# Autodesk Inventor assembly: Lift Assembly Right
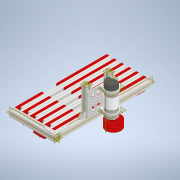
[picture p0: Inventor's stored thumbnail of the model, 180x180]
Saved by Autodesk Inventor 2020 (Build 240168000, 168)
## iProperties
Created: 2019-12-26
Part Number: Lift Assembly Right
Document SubType Name: Assembly
Designer: ball
Author: ball
## Documents named in this file (14)
- D:\FTC8863\2019 Robot\Delivery\Lift Right\Lift Assembly Right.iam
- D:\FTC8863\2019 Robot\Delivery\Lift Right\SAR330  x 5 + couplers right.iam
- D:\FTC8863\Actobotics\585 parts\585075.ipt
- D:\FTC8863\Actobotics\565 parts\xrail_3.5in.ipt
- D:\FTC8863\Actobotics\555 parts\555116 assembly.ipt
- D:\FTC8863\Actobotics\585 parts\585721.ipt
- D:\FTC8863\2019 Robot\Delivery\spool double 2 in diameter.iam
- D:\FTC8863\Andymark\am-2964a Neverest Classic 40.ipt
- D:\FTC8863\2019 Robot\Delivery\Lift Right\Limit switch top + mount right.iam
- D:\FTC8863\StepLibraries\Screws\M3 x 25 HEX HEAD CAP SCREW.ipt
- D:\FTC8863\2019 Robot\Delivery\Lift Right\Limit switch bottom + mount right.iam
- D:\FTC8863\Actobotics\585 parts\585071.ipt
- D:\FTC8863\2019 Robot\Delivery\x-rail 6.026 in.ipt
- D:\FTC8863\Actobotics\585 parts\585076.ipt
## Components (18 placed, 13 different names)
1. SAR330  x 5 + couplers right:1 [sub-assembly] — Mate:8, Flush:3, Mate:18, Mate:25, Mate:48, Mate:49, Flush:10, Mate:51, Mate:53, Flush:11, Mate:65, Flush:14, Mate:66, Mate:67, Mate:73, Mate:75, Flush:18
2. x-rail 6.026 in:1 — Mate:8, Flush:3, Mate:54, Mate:55, Mate:68, Mate:69, Mate:70
3. 585075:2
4. xrail_3.5in:2 — Flush:15, Flush:16, Mate:66, Mate:76, Mate:77, Flush:18
5. xrail_3.5in:3 — Mate:18, Mate:25, Mate:56, Flush:12, Mate:57, Flush:16, Mate:74, Flush:17
6. 585721:1 — Mate:57, Mate:58, Flush:13, Mate:59, Mate:61, Mate:62, Mate:65, Flush:15
7. 585721:2 — Mate:56, Flush:12, Mate:58, Flush:13, Mate:60, Mate:63, Mate:64
8. 555116 assembly:3 — Mate:46, Mate:59, Mate:61, Mate:62
9. 555116 assembly:4 — Mate:60, Mate:63, Mate:64
10. spool double 2 in diameter:1 [sub-assembly] — Flush:14
11. am-2964a Neverest Classic 40:1 — Mate:46
12. Limit switch top + mount right:1 [sub-assembly] — Mate:48, Mate:49, Flush:10, Mate:50, Mate:52
13. M3 x 25 HEX HEAD CAP SCREW:1 — Mate:50, Mate:51
14. M3 x 25 HEX HEAD CAP SCREW:2 — Mate:52, Mate:53
15. Limit switch bottom + mount right:1 [sub-assembly] — Mate:54, Mate:55, Flush:11
16. 585071:1 — Mate:75, Mate:76, Mate:77
17. 585071:2 — Mate:73, Mate:74, Flush:17
18. 585076:1 — Mate:67, Mate:68, Mate:69, Mate:70
## Relationships (46: Mate 36, Flush 10)
- [Mate]: x-rail 6.026 in:1 ↔ 585075:2
- [Mate]: x-rail 6.026 in:1 ↔ 585075:2
- Mate:8: SAR330  x 5 + couplers right:1 ↔ x-rail 6.026 in:1
- Flush:3: SAR330  x 5 + couplers right:1 ↔ x-rail 6.026 in:1
- Mate:18: SAR330  x 5 + couplers right:1 ↔ xrail_3.5in:3
- Mate:25: SAR330  x 5 + couplers right:1 ↔ xrail_3.5in:3
- [Mate]: spool double 2 in diameter:1 ↔ am-2964a Neverest Classic 40:1
- [Mate]: spool double 2 in diameter:1 ↔ am-2964a Neverest Classic 40:1
- Mate:46: 555116 assembly:3 ↔ am-2964a Neverest Classic 40:1
- Mate:48: SAR330  x 5 + couplers right:1 ↔ Limit switch top + mount right:1
- Mate:49: SAR330  x 5 + couplers right:1 ↔ Limit switch top + mount right:1
- Flush:10 (2.54 mm): SAR330  x 5 + couplers right:1 ↔ Limit switch top + mount right:1
- Mate:50: Limit switch top + mount right:1 ↔ M3 x 25 HEX HEAD CAP SCREW:1
- Mate:51: SAR330  x 5 + couplers right:1 ↔ M3 x 25 HEX HEAD CAP SCREW:1
- Mate:52: Limit switch top + mount right:1 ↔ M3 x 25 HEX HEAD CAP SCREW:2
- Mate:53: SAR330  x 5 + couplers right:1 ↔ M3 x 25 HEX HEAD CAP SCREW:2
- Mate:54: x-rail 6.026 in:1 ↔ Limit switch bottom + mount right:1
- Mate:55: x-rail 6.026 in:1 ↔ Limit switch bottom + mount right:1
- Flush:11: SAR330  x 5 + couplers right:1 ↔ Limit switch bottom + mount right:1
- Mate:56: xrail_3.5in:3 ↔ 585721:2
- Flush:12: xrail_3.5in:3 ↔ 585721:2
- Mate:57: xrail_3.5in:3 ↔ 585721:1
- Mate:58: 585721:1 ↔ 585721:2
- Flush:13: 585721:1 ↔ 585721:2
- Mate:59: 585721:1 ↔ 555116 assembly:3
- Mate:60: 585721:2 ↔ 555116 assembly:4
- Mate:61: 585721:1 ↔ 555116 assembly:3
- Mate:62: 585721:1 ↔ 555116 assembly:3
- Mate:63: 585721:2 ↔ 555116 assembly:4
- Mate:64: 585721:2 ↔ 555116 assembly:4
- Mate:65: SAR330  x 5 + couplers right:1 ↔ 585721:1
- Flush:14 (-8.0264 mm): SAR330  x 5 + couplers right:1 ↔ spool double 2 in diameter:1
- Flush:15: xrail_3.5in:2 ↔ 585721:1
- Flush:16: xrail_3.5in:2 ↔ xrail_3.5in:3
- Mate:66: SAR330  x 5 + couplers right:1 ↔ xrail_3.5in:2
- Mate:67: SAR330  x 5 + couplers right:1 ↔ 585076:1
- Mate:68: x-rail 6.026 in:1 ↔ 585076:1
- Mate:69: x-rail 6.026 in:1 ↔ 585076:1
- Mate:70: x-rail 6.026 in:1 ↔ 585076:1
- Mate:73: SAR330  x 5 + couplers right:1 ↔ 585071:2
- Mate:74: xrail_3.5in:3 ↔ 585071:2
- Flush:17: xrail_3.5in:3 ↔ 585071:2
- Mate:75: SAR330  x 5 + couplers right:1 ↔ 585071:1
- Mate:76: xrail_3.5in:2 ↔ 585071:1
- Mate:77: xrail_3.5in:2 ↔ 585071:1
- Flush:18 (120.65 mm): SAR330  x 5 + couplers right:1 ↔ xrail_3.5in:2
